# Autodesk Inventor assembly: Line Follower
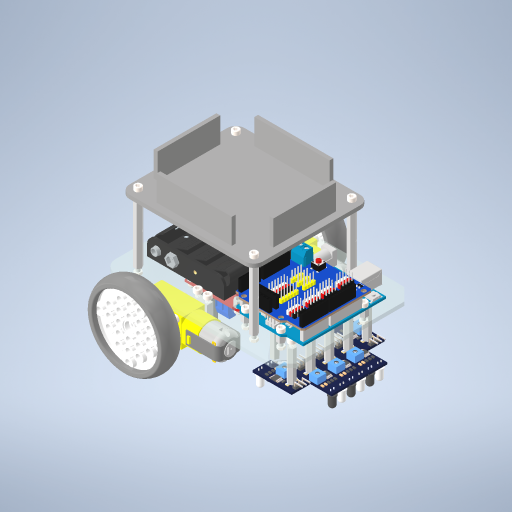
[picture p0: Inventor's stored thumbnail of the model, 512x512]
Saved by Autodesk Inventor 2023 (Build 270158000, 158)
## iProperties
Created: 2022-11-16
Part Number: Line Follower
Document SubType Name: Assembly
Designer: Pyae Htoo Khant
Mass: 330.576 g
Surface Area: 2126.97 cm^2
Volume: 246.45 cm^3
Density: 1.34135 g/cm^3
Author: Pyae Htoo Khant
## Documents named in this file (18)
- C:\Users\Pyae Htoo Khant\Downloads\Line Follower Final\Line Follower.iam
- C:\Users\Pyae Htoo Khant\Downloads\Line Follower Final\arduino uno.iam
- C:\Users\Pyae Htoo Khant\Downloads\Line Follower Final\Motor holder.ipt
- C:\Users\Pyae Htoo Khant\Downloads\Line Follower Final\yellow_toy_motor_dims.ipt
- C:\Users\Pyae Htoo Khant\Downloads\Line Follower Final\L298N Motor Driver.ipt
- C:\Users\Pyae Htoo Khant\Downloads\Line Follower Final\Pole.ipt
- C:\Users\Pyae Htoo Khant\Downloads\Line Follower Final\small pole.ipt
- C:\Users\Pyae Htoo Khant\Downloads\Line Follower Final\Line Follow Update.ipt
- C:\Users\Pyae Htoo Khant\Downloads\Line Follower Final\Caster Ball Wheel (1).iam
- C:\Users\Pyae Htoo Khant\Downloads\Line Follower Final\Line Follow Roof.ipt
- C:\Users\Pyae Htoo Khant\Downloads\Line Follower Final\IR Sensor.ipt
- C:\Users\Pyae Htoo Khant\Downloads\Line Follower Final\User Library-R6_AA_UM3-1_5V_holder4AA.ipt
- C:\Users\Pyae Htoo Khant\Downloads\Line Follower Final\Plastic Timing Pulley 90T For Motor.ipt
- C:\Users\Pyae Htoo Khant\Downloads\Line Follower Final\Tire 90T B.ipt
- C:\Users\Pyae Htoo Khant\Downloads\Line Follower Final\Arduino Sensor Board V1.ipt
- C:\Users\Pyae Htoo Khant\Documents\Line Follower Final\M3x6.ipt
- C:\Users\Pyae Htoo Khant\Documents\Line Follower Final\M3 nut.ipt
- C:\Users\Pyae Htoo Khant\Documents\Line Follower Final\M3x25.ipt
## Components (89 placed, 17 different names)
1. arduino uno:1 [sub-assembly] — Rigid:18, Rigid:47, Rigid:48, Rotational:3, Rigid:62, Insert:33, Insert:34, Insert:35, Insert:36
2. Motor holder:1 — Rigid:7, Rigid:50, Insert:42, Insert:45
3. Motor holder:2 — Rigid:6, Rigid:51, Insert:43, Insert:44
4. yellow_toy_motor_dims:2 — Rigid:6, Rotational:32, Insert:40, Insert:41
5. yellow_toy_motor_dims:3 — Rigid:7, Rotational:33, Insert:38, Insert:39
6. L298N Motor Driver:1 — Rigid:33, Insert:27, Insert:28, Insert:37
7. Pole:1 — Rigid:9, Rigid:59
8. Pole:2 — Rigid:9
9. Pole:3 — Rigid:35, Rigid:36
10. Pole:11 — Rigid:60
11. Pole:12
12. Pole:13 — Rigid:55
13. Pole:14
14. Pole:15 — Rigid:58
15. Pole:16 — Rigid:61
16. small pole:1 — Rotational:3
17. small pole:2 — Rigid:48
18. small pole:3 — Rigid:57
19. small pole:4 — Rigid:47, Rigid:49
20. small pole:5 — Rigid:32, Insert:25
21. small pole:6 — Rigid:31, Rigid:33
22. small pole:7 — Rigid:56
23. small pole:8 — Rigid:18
24. Line Follow Update:1 — Rigid:34, Rigid:31, Rigid:32, Rigid:36, Rigid:41, Rigid:42, Rigid:44, Rigid:45, Rigid:46, Rigid:49, Rigid:50, Rigid:51, Rigid:55, Rigid:56, Rigid:57, Rigid:58, Rigid:59, Rigid:60, Insert:6, Insert:7, Insert:8, Insert:9, Insert:10, Insert:11, Insert:12, Insert:13, Insert:14, Insert:22, Insert:23, Insert:24, Insert:26, Insert:29, Insert:30, Insert:31, Insert:32
25. Line Follow Roof:1 — Rigid:61, Insert:3, Insert:4, Insert:5, Insert:46
26. Pole:17 — Insert:20
27. Pole:18 — Rotational:31, Rigid:34, Insert:21
28. Caster Ball Wheel (1):3 [sub-assembly] — Rotational:31
29. IR Sensor:1 — Rigid:35, Insert:15
30. Pole:19 — Rigid:46
31. IR Sensor:2 — Insert:18
32. Pole:20 — Rigid:42
33. IR Sensor:3 — Insert:17
34. Pole:21 — Rigid:39, Rigid:45
35. IR Sensor:4 — Rigid:39, Insert:19
36. Pole:22 — Rigid:41
37. IR Sensor:5 — Insert:16
38. User Library-R6_AA_UM3-1_5V_holder4AA:1 — Rigid:44
39. Plastic Timing Pulley 90T For Motor:2 — Insert:1, Rotational:33
40. Tire 90T B:2 — Insert:1
41. Plastic Timing Pulley 90T For Motor:3 — Rotational:32
42. Tire 90T B:3
43. Arduino Sensor Board V1:1 — Rigid:62
44. M3x6:1 — Insert:3
45. M3x6:2 — Insert:46
46. M3x6:3 — Insert:5
47. M3x6:4 — Insert:4
48. M3x6:5 — Insert:9
49. M3x6:6 — Insert:10
50. M3x6:7 — Insert:7
51. M3x6:8 — Insert:8
52. M3x6:9 — Insert:6
53. M3x6:10 — Insert:13
54. M3x6:11 — Insert:12
55. M3x6:12 — Insert:11
56. M3x6:13 — Insert:14
57. M3 nut:1 — Insert:16
58. M3 nut:2 — Insert:15
59. M3 nut:3 — Insert:18
60. M3 nut:4 — Insert:19
61. M3 nut:5 — Insert:17
62. M3 nut:6 — Insert:26
63. M3 nut:7 — Insert:20
64. M3 nut:8 — Insert:21
65. M3 nut:9 — Insert:24
66. M3 nut:10 — Insert:25
67. M3 nut:11 — Insert:22
68. M3 nut:12 — Insert:23
69. M3 nut:13 — Insert:28
70. M3 nut:14 — Insert:30
71. M3 nut:15 — Insert:27
72. M3 nut:16 — Insert:31
73. M3 nut:17 — Insert:29
74. M3 nut:18
75. M3 nut:19 — Insert:32
76. M3x6:15 — Insert:36
77. M3x6:16 — Insert:34
78. M3x6:17 — Insert:33
79. M3x6:18 — Insert:35
80. M3 nut:20
81. M3 nut:21 — Insert:37
82. M3x25:1 — Insert:40
83. M3x25:2 — Insert:39
84. M3x25:3 — Insert:38
85. M3x25:4 — Insert:41
86. M3 nut:22 — Insert:42
87. M3 nut:23 — Insert:43
88. M3 nut:24 — Insert:44
89. M3 nut:25 — Insert:45
## Relationships (86: Insert 46, WeldJoint 36, RevoluteJoint 4)
- Rigid:6 [WeldJoint]: Motor holder:2 ↔ yellow_toy_motor_dims:2
- Rigid:7 [WeldJoint]: Motor holder:1 ↔ yellow_toy_motor_dims:3
- Rigid:9 [WeldJoint]: Pole:1 ↔ Pole:2
- [WeldJoint]: Pole:11 ↔ Pole:12
- [WeldJoint]: Pole:13 ↔ Pole:14
- [WeldJoint]: Pole:15 ↔ Pole:16
- Rigid:18 [WeldJoint]: arduino uno:1 ↔ small pole:8
- [WeldJoint]: Pole:17 ↔ Caster Ball Wheel (1):3
- Rotational:31 [RevoluteJoint]: Pole:18 ↔ Caster Ball Wheel (1):3
- Rigid:34 [WeldJoint]: Line Follow Update:1 ↔ Pole:18
- Rigid:31 [WeldJoint]: small pole:6 ↔ Line Follow Update:1
- Rigid:32 [WeldJoint]: small pole:5 ↔ Line Follow Update:1
- Rigid:33 [WeldJoint]: L298N Motor Driver:1 ↔ small pole:6
- Rigid:35 [WeldJoint]: Pole:3 ↔ IR Sensor:1
- Rigid:36 [WeldJoint]: Pole:3 ↔ Line Follow Update:1
- [WeldJoint]: Pole:19 ↔ IR Sensor:2
- [WeldJoint]: Pole:20 ↔ IR Sensor:3
- Rigid:39 [WeldJoint]: Pole:21 ↔ IR Sensor:4
- [WeldJoint]: Pole:22 ↔ IR Sensor:5
- Rigid:41 [WeldJoint]: Line Follow Update:1 ↔ Pole:22
- Rigid:42 [WeldJoint]: Line Follow Update:1 ↔ Pole:20
- Rigid:44 [WeldJoint]: Line Follow Update:1 ↔ User Library-R6_AA_UM3-1_5V_holder4AA:1
- Rigid:45 [WeldJoint]: Line Follow Update:1 ↔ Pole:21
- Rigid:46 [WeldJoint]: Line Follow Update:1 ↔ Pole:19
- Rigid:47 [WeldJoint]: arduino uno:1 ↔ small pole:4
- Rigid:48 [WeldJoint]: arduino uno:1 ↔ small pole:2
- Rotational:3 [RevoluteJoint]: arduino uno:1 ↔ small pole:1
- Rigid:49 [WeldJoint]: small pole:4 ↔ Line Follow Update:1
- Rigid:50 [WeldJoint]: Motor holder:1 ↔ Line Follow Update:1
- Rigid:51 [WeldJoint]: Motor holder:2 ↔ Line Follow Update:1
- Rigid:55 [WeldJoint]: Pole:13 ↔ Line Follow Update:1
- Rigid:56 [WeldJoint]: small pole:7 ↔ Line Follow Update:1
- Rigid:57 [WeldJoint]: small pole:3 ↔ Line Follow Update:1
- Rigid:58 [WeldJoint]: Pole:15 ↔ Line Follow Update:1
- Rigid:59 [WeldJoint]: Pole:1 ↔ Line Follow Update:1
- Rigid:60 [WeldJoint]: Pole:11 ↔ Line Follow Update:1
- Rigid:61 [WeldJoint]: Pole:16 ↔ Line Follow Roof:1
- Insert:1: Plastic Timing Pulley 90T For Motor:2 ↔ Tire 90T B:2
- [Insert]: Plastic Timing Pulley 90T For Motor:3 ↔ Tire 90T B:3
- Rotational:32 [RevoluteJoint]: yellow_toy_motor_dims:2 ↔ Plastic Timing Pulley 90T For Motor:3
- Rotational:33 [RevoluteJoint]: yellow_toy_motor_dims:3 ↔ Plastic Timing Pulley 90T For Motor:2
- Rigid:62 [WeldJoint] (8.5 mm): arduino uno:1 ↔ Arduino Sensor Board V1:1
- Insert:3: Line Follow Roof:1 ↔ M3x6:1
- Insert:4: Line Follow Roof:1 ↔ M3x6:4
- Insert:5: Line Follow Roof:1 ↔ M3x6:3
- Insert:6: Line Follow Update:1 ↔ M3x6:9
- Insert:7: Line Follow Update:1 ↔ M3x6:7
- Insert:8: Line Follow Update:1 ↔ M3x6:8
- Insert:9: Line Follow Update:1 ↔ M3x6:5
- Insert:10: Line Follow Update:1 ↔ M3x6:6
- Insert:11: Line Follow Update:1 ↔ M3x6:12
- Insert:12: Line Follow Update:1 ↔ M3x6:11
- Insert:13: Line Follow Update:1 ↔ M3x6:10
- Insert:14: Line Follow Update:1 ↔ M3x6:13
- Insert:15: IR Sensor:1 ↔ M3 nut:2
- Insert:16: IR Sensor:5 ↔ M3 nut:1
- Insert:17: IR Sensor:3 ↔ M3 nut:5
- Insert:18: IR Sensor:2 ↔ M3 nut:3
- Insert:19: IR Sensor:4 ↔ M3 nut:4
- Insert:20: Pole:17 ↔ M3 nut:7
- Insert:21: Pole:18 ↔ M3 nut:8
- Insert:22: Line Follow Update:1 ↔ M3 nut:11
- Insert:23: Line Follow Update:1 ↔ M3 nut:12
- Insert:24: Line Follow Update:1 ↔ M3 nut:9
- Insert:25 (-3 mm): small pole:5 ↔ M3 nut:10
- Insert:26: Line Follow Update:1 ↔ M3 nut:6
- Insert:27: L298N Motor Driver:1 ↔ M3 nut:15
- Insert:28: L298N Motor Driver:1 ↔ M3 nut:13
- Insert:29: Line Follow Update:1 ↔ M3 nut:17
- Insert:30: Line Follow Update:1 ↔ M3 nut:14
- Insert:31: Line Follow Update:1 ↔ M3 nut:16
- Insert:32: Line Follow Update:1 ↔ M3 nut:19
- Insert:33: arduino uno:1 ↔ M3x6:17
- Insert:34: arduino uno:1 ↔ M3x6:16
- Insert:35: arduino uno:1 ↔ M3x6:18
- Insert:36: arduino uno:1 ↔ M3x6:15
- Insert:37: L298N Motor Driver:1 ↔ M3 nut:21
- Insert:38: yellow_toy_motor_dims:3 ↔ M3x25:3
- Insert:39: yellow_toy_motor_dims:3 ↔ M3x25:2
- Insert:40: yellow_toy_motor_dims:2 ↔ M3x25:1
- Insert:41: yellow_toy_motor_dims:2 ↔ M3x25:4
- Insert:42: Motor holder:1 ↔ M3 nut:22
- Insert:43: Motor holder:2 ↔ M3 nut:23
- Insert:44: Motor holder:2 ↔ M3 nut:24
- Insert:45: Motor holder:1 ↔ M3 nut:25
- Insert:46: Line Follow Roof:1 ↔ M3x6:2
## Named parameters: d20_d19 = 0 mm, d21_d19 = 0 mm, d22_d19 = 0 mm, d61_d57 = 0 mm, d62_d58 = 0 mm, d75_d73 = 0 mm, d76_d73 = 0 mm, d77_d73 = 0 mm, d78_d73 = 0 mm, d110_d109 = 0 mm
